# Autodesk Inventor assembly: Assembly8
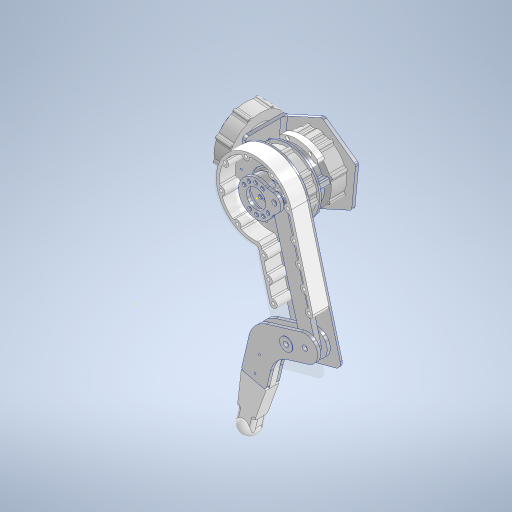
[picture p0: Inventor's stored thumbnail of the model, 512x512]
Saved by Autodesk Inventor 2024.3 (Build 283343000, 343)
## iProperties
Created: 2025-02-12
Part Number: Assembly8
Document SubType Name: Assembly
Designer: 佐藤智貴
Mass: 2204.56 g
Surface Area: 4025.47 cm^2
Volume: 875.413 cm^3
Density: 2.51831 g/cm^3
Author: 佐藤智貴
## Documents named in this file (20)
- C:\Users\佐藤智貴\OneDrive - Chiba Institute of Technology\ドキュメント\Inventor\Biped_robot\Assembly8.iam
- C:\Users\佐藤智貴\OneDrive - Chiba Institute of Technology\ドキュメント\Inventor\Biped_robot\A\BR_parts_08(1).ipt
- C:\Users\佐藤智貴\OneDrive - Chiba Institute of Technology\ドキュメント\Inventor\Biped_robot\A\BR_parts_08(2).ipt
- C:\Users\佐藤智貴\OneDrive - Chiba Institute of Technology\ドキュメント\Inventor\Biped_robot\8108-8.iam
- C:\Users\佐藤智貴\OneDrive - Chiba Institute of Technology\ドキュメント\Inventor\Biped_robot\A\BR_parts_03.ipt
- C:\Users\佐藤智貴\OneDrive - Chiba Institute of Technology\ドキュメント\Inventor\Biped_robot\bearing_MF14mm.ipt
- C:\Users\佐藤智貴\OneDrive - Chiba Institute of Technology\ドキュメント\Inventor\Biped_robot\legparts_01.ipt
- C:\Users\佐藤智貴\OneDrive - Chiba Institute of Technology\ドキュメント\Inventor\Biped_robot\A\BR_parts_07.ipt
- C:\Users\佐藤智貴\OneDrive - Chiba Institute of Technology\ドキュメント\Inventor\Biped_robot\legparts_10.ipt
- C:\Users\佐藤智貴\OneDrive - Chiba Institute of Technology\ドキュメント\Inventor\Biped_robot\A\BR_parts_02.ipt
- C:\Users\佐藤智貴\OneDrive - Chiba Institute of Technology\ドキュメント\Inventor\Biped_robot\A\BR_parts_04_2.ipt
- C:\Users\佐藤智貴\OneDrive - Chiba Institute of Technology\ドキュメント\Inventor\Biped_robot\Hinge_pin15mm.ipt
- C:\Users\佐藤智貴\OneDrive - Chiba Institute of Technology\ドキュメント\Inventor\Biped_robot\BR_parts_06(1).ipt
- C:\Users\佐藤智貴\OneDrive - Chiba Institute of Technology\ドキュメント\Inventor\Biped_robot\BR_parts_06(2).ipt
- C:\Users\佐藤智貴\OneDrive - Chiba Institute of Technology\ドキュメント\Inventor\Biped_robot\Assembly8\AIP\FEA\ez06f8bk0.fins
- C:\Users\佐藤智貴\OneDrive - Chiba Institute of Technology\ドキュメント\Inventor\Biped_robot\Assembly8\AIP\FEA\ez06f8bk0.fsat
- C:\Users\佐藤智貴\OneDrive - Chiba Institute of Technology\ドキュメント\Inventor\Biped_robot\Assembly8\AIP\FEA\ez06f8bk0.ftes
- C:\Users\佐藤智貴\OneDrive - Chiba Institute of Technology\ドキュメント\Inventor\Biped_robot\Assembly8\AIP\FEA\ez06f8bk0.fwiz
- C:\Users\佐藤智貴\OneDrive - Chiba Institute of Technology\ドキュメント\Inventor\Biped_robot\Assembly8\AIP\FEA\ez06f8bts.fmsh
- C:\Users\佐藤智貴\OneDrive - Chiba Institute of Technology\ドキュメント\Inventor\Biped_robot\Assembly8\AIP\FEA\ez06f8btt.fres
## Components (23 placed, 13 different names)
1. BR_parts_08(1):1 — 挿入:1, 挿入:2, 挿入:56, 挿入:77
2. BR_parts_08(2):1 — 挿入:1, 挿入:2, 挿入:21, 挿入:22
3. 8108-8:1 [sub-assembly] — 挿入:44, 挿入:45, 挿入:46, 挿入:47, 挿入:56
4. bearing_MF14mm:1 — 挿入:48, 挿入:49
5. bearing_MF14mm:2 — 挿入:50
6. bearing_MF14mm:3 — 挿入:52, 挿入:76
7. bearing_MF14mm:4 — 挿入:51
8. BR_parts_08(1):2 — 挿入:21, 挿入:22
9. 8108-8:2 [sub-assembly] — 挿入:30, 挿入:31, 挿入:32, 挿入:39, 挿入:40, 挿入:41, 挿入:42
10. 8108-8:3 [sub-assembly] — 挿入:33, 挿入:34
11. legparts_01:1 — 挿入:30, 挿入:46, 挿入:47
12. BR_parts_07:1 — 挿入:31, 挿入:32, 挿入:33, 挿入:34
13. legparts_10:1 — 挿入:39, 挿入:42
14. legparts_10:2 — 挿入:40, 挿入:41
15. BR_parts_02:1 — 挿入:44, 挿入:45, 挿入:48, 挿入:60, 挿入:61, 挿入:63
16. BR_parts_03:1 — 挿入:49, 挿入:50, 挿入:51, 挿入:52
17. BR_parts_04_2:1 — 挿入:60, 挿入:61
18. Hinge_pin15mm:1 — 挿入:63
19. BR_parts_06(1):1 — 挿入:69, 挿入:72, 挿入:75
20. BR_parts_06(1):2 — 挿入:67, 挿入:68, 挿入:71, 挿入:73, 挿入:74, 挿入:76
21. BR_parts_06(2):1 — 挿入:67, 挿入:68, 挿入:69, 挿入:72, 挿入:73, 挿入:74
22. bearing_MF14mm:7 — 挿入:71, 挿入:77
23. bearing_MF14mm:8 — 挿入:75
## Relationships (36: Insert 36)
- 挿入:1 [Insert]: BR_parts_08(1):1 ↔ BR_parts_08(2):1
- 挿入:2 [Insert]: BR_parts_08(1):1 ↔ BR_parts_08(2):1
- 挿入:21 [Insert]: BR_parts_08(2):1 ↔ BR_parts_08(1):2
- 挿入:22 [Insert]: BR_parts_08(2):1 ↔ BR_parts_08(1):2
- 挿入:30 [Insert]: 8108-8:2 ↔ legparts_01:1
- 挿入:31 [Insert]: 8108-8:2 ↔ BR_parts_07:1
- 挿入:32 [Insert]: 8108-8:2 ↔ BR_parts_07:1
- 挿入:33 [Insert]: 8108-8:3 ↔ BR_parts_07:1
- 挿入:34 [Insert]: 8108-8:3 ↔ BR_parts_07:1
- 挿入:39 [Insert]: 8108-8:2 ↔ legparts_10:1
- 挿入:40 [Insert]: 8108-8:2 ↔ legparts_10:2
- 挿入:41 [Insert]: 8108-8:2 ↔ legparts_10:2
- 挿入:42 [Insert]: 8108-8:2 ↔ legparts_10:1
- 挿入:44 [Insert]: 8108-8:1 ↔ BR_parts_02:1
- 挿入:45 [Insert]: 8108-8:1 ↔ BR_parts_02:1
- 挿入:46 [Insert]: 8108-8:1 ↔ legparts_01:1
- 挿入:47 [Insert]: 8108-8:1 ↔ legparts_01:1
- 挿入:48 [Insert] (0.2 mm): bearing_MF14mm:1 ↔ BR_parts_02:1
- 挿入:49 [Insert]: bearing_MF14mm:1 ↔ BR_parts_03:1
- 挿入:50 [Insert]: bearing_MF14mm:2 ↔ BR_parts_03:1
- 挿入:51 [Insert]: bearing_MF14mm:4 ↔ BR_parts_03:1
- 挿入:52 [Insert]: bearing_MF14mm:3 ↔ BR_parts_03:1
- 挿入:56 [Insert]: BR_parts_08(1):1 ↔ 8108-8:1
- 挿入:60 [Insert]: BR_parts_02:1 ↔ BR_parts_04_2:1
- 挿入:61 [Insert]: BR_parts_02:1 ↔ BR_parts_04_2:1
- 挿入:63 [Insert]: BR_parts_02:1 ↔ Hinge_pin15mm:1
- 挿入:67 [Insert]: BR_parts_06(1):2 ↔ BR_parts_06(2):1
- 挿入:68 [Insert]: BR_parts_06(1):2 ↔ BR_parts_06(2):1
- 挿入:69 [Insert]: BR_parts_06(1):1 ↔ BR_parts_06(2):1
- 挿入:71 [Insert]: BR_parts_06(1):2 ↔ bearing_MF14mm:7
- 挿入:72 [Insert]: BR_parts_06(1):1 ↔ BR_parts_06(2):1
- 挿入:73 [Insert]: BR_parts_06(1):2 ↔ BR_parts_06(2):1
- 挿入:74 [Insert]: BR_parts_06(1):2 ↔ BR_parts_06(2):1
- 挿入:75 [Insert]: BR_parts_06(1):1 ↔ bearing_MF14mm:8
- 挿入:76 [Insert] (0.2 mm): bearing_MF14mm:3 ↔ BR_parts_06(1):2
- 挿入:77 [Insert] (1.7 mm): BR_parts_08(1):1 ↔ bearing_MF14mm:7
## Named parameters: sa_0 = 0, sa_1 = -5000, sa_2 = 0, sa_3 = 0, sa_4 = -5000, sa_5 = 0, sa_6 = 0, sa_7 = -5000, sa_8 = 0
note: some values were not read from the file. Shown as the stored number, unit unknown: "sa_0", "sa_1", "sa_2", "sa_3", "sa_4", "sa_5", "sa_6", "sa_7", "sa_8".
